# Autodesk Inventor assembly: ASSEMBLY_pring_vbar_holder
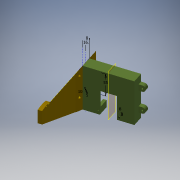
[picture p0: Inventor's stored thumbnail of the model, 180x180]
Saved by Autodesk Inventor 2018 (Build 220112000, 112)
## iProperties
Created: 2026-06-13
Part Number: ASSEMBLY_pring_vbar_holder
Document SubType Name: Assembly
Designer: neo
Author: neo
## Documents named in this file (4)
- C:\Users\neo\Documents\neoatlantis-shared\projects\kreion\design2\ASSEMBLY_pring_vbar_holder.iam
- C:\Users\neo\Documents\neoatlantis-shared\projects\kreion\design2\PRING_vertical_bar.ipt
- C:\Users\neo\Documents\neoatlantis-shared\projects\kreion\design2\PRING_piston_holder_half.ipt
- C:\Users\neo\Documents\neoatlantis-shared\projects\kreion\design2\HELP_ROD_D4x100.ipt
## Components (4 placed, 3 different names)
1. PRING_vertical_bar:1 — Mate:2, Mate:6, Tangent:5
2. PRING_piston_holder_half:1 — Mate:2, Tangent:2, Tangent:3, Mate:4, Mate:5, Tangent:4, Mate:6, Tangent:5
3. HELP_ROD_D4x100:1 — Tangent:3, Mate:4
4. HELP_ROD_D4x100:2 — Tangent:2, Mate:5, Tangent:4
## Relationships (8: Mate 4, Tangent 4)
- Mate:2: PRING_vertical_bar:1 ↔ PRING_piston_holder_half:1
- Tangent:2: PRING_piston_holder_half:1 ↔ HELP_ROD_D4x100:2
- Tangent:3: PRING_piston_holder_half:1 ↔ HELP_ROD_D4x100:1
- Mate:4: PRING_piston_holder_half:1 ↔ HELP_ROD_D4x100:1
- Mate:5: PRING_piston_holder_half:1 ↔ HELP_ROD_D4x100:2
- Tangent:4: PRING_piston_holder_half:1 ↔ HELP_ROD_D4x100:2
- Mate:6: PRING_vertical_bar:1 ↔ PRING_piston_holder_half:1
- Tangent:5: PRING_vertical_bar:1 ↔ PRING_piston_holder_half:1
